# Autodesk Inventor assembly: Y
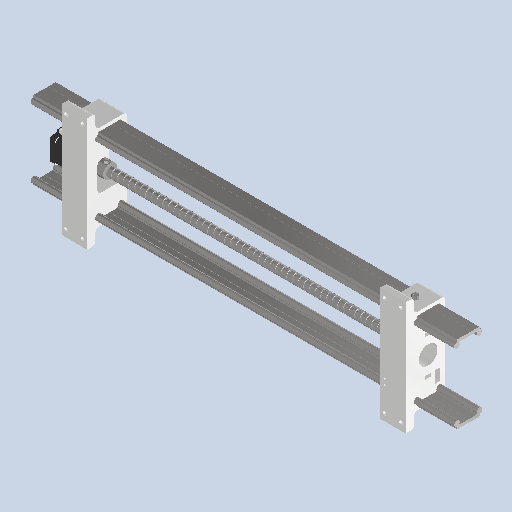
[picture p0: Inventor's stored thumbnail of the model, 512x512]
Saved by Autodesk Inventor 2024 (Build 280153000, 153)
## iProperties
Created: 2022-04-26
Part Number: Y
Document SubType Name: Assembly
Designer: mikoma
Author: mikoma
## Documents named in this file (14)
- D:\@home\mikoma\Dokumenty\DR\CartesianRobotsDigitalTwin\model\Workspaces\Obszar roboczy\assembly_v3\X\X.iam
- D:\@home\mikoma\Dokumenty\DR\CartesianRobotsDigitalTwin\model\Workspaces\Obszar roboczy\assembly_v3\X\XMotorMount.ipt
- D:\@home\mikoma\Dokumenty\DR\CartesianRobotsDigitalTwin\model\Workspaces\Obszar roboczy\assembly_v3\X\WS_10_40_X.ipt
- D:\@home\mikoma\Dokumenty\DR\CartesianRobotsDigitalTwin\model\Workspaces\Obszar roboczy\assembly_v3\X\XFloating.ipt
- D:\@home\mikoma\Dokumenty\DR\CartesianRobotsDigitalTwin\model\Workspaces\Obszar roboczy\content\nema17\Nema17 Stepper Motor.ipt
- D:\@home\mikoma\Dokumenty\DR\CartesianRobotsDigitalTwin\model\Workspaces\Obszar roboczy\content\manipulatorSharedParts\Cartesian1_BallScrew.ipt
- D:\@home\mikoma\Dokumenty\DR\CartesianRobotsDigitalTwin\model\Workspaces\Obszar roboczy\content\manipulatorSharedParts\Cartesian2_BallBearing_25x37x7.ipt
- D:\@home\mikoma\Dokumenty\DR\CartesianRobotsDigitalTwin\model\Workspaces\Obszar roboczy\content\manipulatorSharedParts\Cartesian1_12_12_Clutch.ipt
- D:\@home\mikoma\Dokumenty\DR\CartesianRobotsDigitalTwin\model\Workspaces\Obszar roboczy\content\manipulatorSharedParts\endCup.ipt
- D:\@home\mikoma\Dokumenty\DR\CartesianRobotsDigitalTwin\model\Workspaces\Obszar roboczy\content\manipulatorSharedParts\stopSw.ipt
- D:\@home\mikoma\Dokumenty\DR\CartesianRobotsDigitalTwin\model\Workspaces\Obszar roboczy\content\manipulatorSharedParts\Connector_female.ipt
- D:\@home\mikoma\Dokumenty\DR\CartesianRobotsDigitalTwin\model\Workspaces\Obszar roboczy\CC\pl-PL\ISO 4762(1)\DIN EN ISO 4762 - M6 x 60.ipt
- D:\@home\mikoma\Dokumenty\DR\CartesianRobotsDigitalTwin\model\Workspaces\Obszar roboczy\CC\pl-PL\DIN 7984\DIN 7984 - M3 x 18.ipt
- D:\@home\mikoma\Dokumenty\DR\CartesianRobotsDigitalTwin\model\Workspaces\Obszar roboczy\CC\pl-PL\ISO 4032(2)\ISO 4032 - M6 - ISO.ipt
## Components (19 placed, 13 different names)
1. XMotorMount:1 — Zestawiające:1, Równoległe:1, Zestawiające:2, Zestawiające:17, Zestawiające:18, Zestawiające:19, Kątowe:1, Zestawiające:39, Zestawiające:40, Zestawiające:41, Zestawiające:42, Zestawiające:43, Zestawiające:44, Zestawiające:45, Równoległe:6, Równoległe:7, Zestawiające:46, Zestawiające:57, Zestawiające:58, Zestawiające:59, Zestawiające:60, Zestawiające:61, Zestawiające:62, Zestawiające:63, Zestawiające:64
2. WS_10_40_X:1 — Zestawiające:9, Zestawiające:43, Zestawiające:44, Równoległe:7
3. WS_10_40_X:2 — Zestawiające:10, Zestawiające:42, Zestawiające:45, Równoległe:6
4. XFloating:1 — Zestawiające:9, Zestawiające:10, Zestawiające:24, Zestawiające:25, Zestawiające:49, Zestawiające:50, Zestawiające:51, Zestawiające:53, Zestawiające:54, Zestawiające:55, Zestawiające:56, Kątowe:2, Zestawiające:66, Zestawiające:68, Kątowe:3
5. Nema17 Stepper Motor:1 — Zestawiające:17, Zestawiające:18, Kątowe:1
6. Ball Screw:1 — Zestawiające:20, Zestawiające:21, Zestawiające:52
7. Ball Bearing 25x37x7:1 — Zestawiające:24, Zestawiające:25, Zestawiające:47, Zestawiające:48
8. Clutch — Zestawiające:19, Zestawiające:20, Zestawiające:21, Zestawiające:46
9. endCup:1 — Zestawiające:47, Zestawiające:48, Zestawiające:52
10. Connector_female:1 — Zestawiające:39, Zestawiające:40, Zestawiające:41
11. stopSw:2 — Zestawiające:49, Zestawiające:50, Zestawiające:51
12. ISO 4032 M6:1 — Zestawiające:65, Kątowe:2, Zestawiające:66
13. ISO 4032 M6:2 — Zestawiające:67, Zestawiające:68, Kątowe:3
14. DIN 7984 M3 x 18:4 — Zestawiające:60, Zestawiające:64
15. DIN 7984 M3 x 18:3 — Zestawiające:59, Zestawiające:63
16. DIN 7984 M3 x 18:2 — Zestawiające:58, Zestawiające:62
17. DIN 7984 M3 x 18:1 — Zestawiające:57, Zestawiające:61
18. DIN EN ISO 4762 M6 x 60:2 — Zestawiające:55, Zestawiające:56, Zestawiające:65
19. DIN EN ISO 4762 M6 x 60:1 — Zestawiające:53, Zestawiające:54, Zestawiające:67
## Relationships (47: Mate 41, Flush 3, Angle 3)
- Zestawiające:1 [Mate]: XMotorMount:1
- Równoległe:1 [Flush]: XMotorMount:1
- Zestawiające:2 [Mate]: XMotorMount:1
- Zestawiające:9 [Mate]: WS_10_40_X:1 ↔ XFloating:1
- Zestawiające:10 [Mate]: WS_10_40_X:2 ↔ XFloating:1
- Zestawiające:17 [Mate]: XMotorMount:1 ↔ Nema17 Stepper Motor:1
- Zestawiające:18 [Mate]: XMotorMount:1 ↔ Nema17 Stepper Motor:1
- Zestawiające:19 [Mate]: XMotorMount:1 ↔ Clutch
- Zestawiające:20 [Mate]: Ball Screw:1 ↔ Clutch
- Zestawiające:21 [Mate]: Ball Screw:1 ↔ Clutch
- Zestawiające:24 [Mate]: XFloating:1 ↔ Ball Bearing 25x37x7:1
- Zestawiające:25 [Mate]: XFloating:1 ↔ Ball Bearing 25x37x7:1
- Kątowe:1 [Angle] (0 deg): XMotorMount:1 ↔ Nema17 Stepper Motor:1
- Zestawiające:39 [Mate]: XMotorMount:1 ↔ Connector_female:1
- Zestawiające:40 [Mate]: XMotorMount:1 ↔ Connector_female:1
- Zestawiające:41 [Mate]: XMotorMount:1 ↔ Connector_female:1
- Zestawiające:42 [Mate]: XMotorMount:1 ↔ WS_10_40_X:2
- Zestawiające:43 [Mate]: XMotorMount:1 ↔ WS_10_40_X:1
- Zestawiające:44 [Mate]: XMotorMount:1 ↔ WS_10_40_X:1
- Zestawiające:45 [Mate]: XMotorMount:1 ↔ WS_10_40_X:2
- Równoległe:6 [Flush] (-70 mm): XMotorMount:1 ↔ WS_10_40_X:2
- Równoległe:7 [Flush] (-70 mm): XMotorMount:1 ↔ WS_10_40_X:1
- Zestawiające:46 [Mate]: XMotorMount:1 ↔ Clutch
- Zestawiające:47 [Mate]: Ball Bearing 25x37x7:1 ↔ endCup:1
- Zestawiające:48 [Mate]: Ball Bearing 25x37x7:1 ↔ endCup:1
- Zestawiające:49 [Mate]: XFloating:1 ↔ stopSw:2
- Zestawiające:50 [Mate]: XFloating:1 ↔ stopSw:2
- Zestawiające:51 [Mate]: XFloating:1 ↔ stopSw:2
- Zestawiające:52 [Mate]: Ball Screw:1 ↔ endCup:1
- Zestawiające:53 [Mate]: XFloating:1 ↔ DIN EN ISO 4762 M6 x 60:1
- Zestawiające:54 [Mate]: XFloating:1 ↔ DIN EN ISO 4762 M6 x 60:1
- Zestawiające:55 [Mate]: XFloating:1 ↔ DIN EN ISO 4762 M6 x 60:2
- Zestawiające:56 [Mate]: XFloating:1 ↔ DIN EN ISO 4762 M6 x 60:2
- Zestawiające:57 [Mate]: XMotorMount:1 ↔ DIN 7984 M3 x 18:1
- Zestawiające:58 [Mate]: XMotorMount:1 ↔ DIN 7984 M3 x 18:2
- Zestawiające:59 [Mate]: XMotorMount:1 ↔ DIN 7984 M3 x 18:3
- Zestawiające:60 [Mate]: XMotorMount:1 ↔ DIN 7984 M3 x 18:4
- Zestawiające:61 [Mate]: XMotorMount:1 ↔ DIN 7984 M3 x 18:1
- Zestawiające:62 [Mate]: XMotorMount:1 ↔ DIN 7984 M3 x 18:2
- Zestawiające:63 [Mate]: XMotorMount:1 ↔ DIN 7984 M3 x 18:3
- Zestawiające:64 [Mate]: XMotorMount:1 ↔ DIN 7984 M3 x 18:4
- Zestawiające:65 [Mate]: ISO 4032 M6:1 ↔ DIN EN ISO 4762 M6 x 60:2
- Kątowe:2 [Angle] (0 deg): XFloating:1 ↔ ISO 4032 M6:1
- Zestawiające:66 [Mate]: XFloating:1 ↔ ISO 4032 M6:1
- Zestawiające:67 [Mate]: ISO 4032 M6:2 ↔ DIN EN ISO 4762 M6 x 60:1
- Zestawiające:68 [Mate]: XFloating:1 ↔ ISO 4032 M6:2
- Kątowe:3 [Angle] (0 deg): XFloating:1 ↔ ISO 4032 M6:2
